# Autodesk Inventor assembly: Assembly3
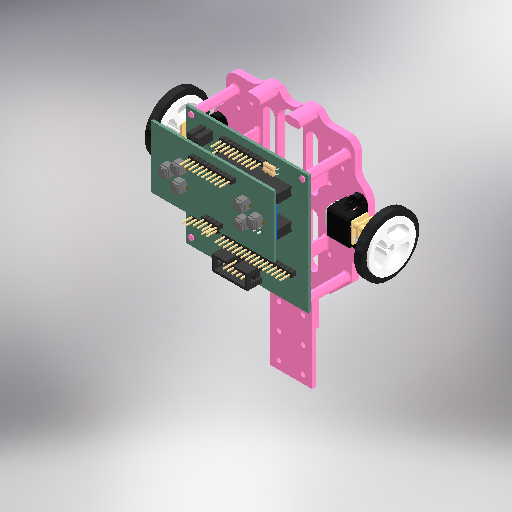
[picture p0: Inventor's stored thumbnail of the model, 512x512]
Saved by Autodesk Inventor 2025.2 (Build 292293000, 293)
## iProperties
Created: 2025-11-09
Part Number: Assembly3
Document SubType Name: Assembly
Designer: ia088
Author: ia088
## Documents named in this file (7)
- C:\Users\ia088\OneDrive\Dokumen\Prak.Robotika\board fix\Assembly3.iam
- C:\Users\ia088\OneDrive\Dokumen\Prak.Robotika\board fix\BASE_LF.ipt
- C:\Users\ia088\OneDrive\Dokumen\Prak.Robotika\board fix\motor.iam
- C:\Users\ia088\OneDrive\Dokumen\Prak.Robotika\board fix\SENSOR_3D1.iam
- C:\Users\ia088\OneDrive\Dokumen\Prak.Robotika\board fix\main_board1\main_board1\main_board1.iam
- C:\Users\ia088\OneDrive\Dokumen\Prak.Robotika\board fix\board_ctrl\board_ctrl\board_ctrl.iam
- C:\Users\ia088\OneDrive\Dokumen\Prak.Robotika\board fix\Arduino Nano\Arduino Nano\Arduino Nano.iam
## Components (7 placed, 6 different names)
1. motor:1 [sub-assembly] — Mate:4, Mate:5, Mate:6
2. motor:2 [sub-assembly] — Mate:1, Mate:2, Mate:3
3. BASE_LF:1 — Mate:1, Mate:2, Mate:3, Mate:4, Mate:5, Mate:6, Mate:7, Mate:8, Mate:9, Mate:10, Mate:11, Mate:12, Mate:13
4. SENSOR_3D1:1 [sub-assembly] — Mate:7, Mate:8, Mate:9
5. main_board1:1 [sub-assembly] — Mate:10, Mate:11, Mate:12, Mate:13, Mate:14, Flush:1, Flush:2, Flush:3, Flush:4
6. board_ctrl:1 [sub-assembly] — Mate:15, Flush:3, Flush:4
7. Arduino Nano:1 [sub-assembly] — Mate:14, Flush:1, Flush:2, Mate:15
## Relationships (19: Mate 15, Flush 4)
- Mate:1: motor:2 ↔ BASE_LF:1
- Mate:2: motor:2 ↔ BASE_LF:1
- Mate:3: motor:2 ↔ BASE_LF:1
- Mate:4: motor:1 ↔ BASE_LF:1
- Mate:5: motor:1 ↔ BASE_LF:1
- Mate:6: motor:1 ↔ BASE_LF:1
- Mate:7: BASE_LF:1 ↔ SENSOR_3D1:1
- Mate:8: BASE_LF:1 ↔ SENSOR_3D1:1
- Mate:9: BASE_LF:1 ↔ SENSOR_3D1:1
- Mate:10: BASE_LF:1 ↔ main_board1:1
- Mate:11: BASE_LF:1 ↔ main_board1:1
- Mate:12: BASE_LF:1 ↔ main_board1:1
- Mate:13: BASE_LF:1 ↔ main_board1:1
- Mate:14: main_board1:1 ↔ Arduino Nano:1
- Flush:1: main_board1:1 ↔ Arduino Nano:1
- Flush:2: main_board1:1 ↔ Arduino Nano:1
- Mate:15: board_ctrl:1 ↔ Arduino Nano:1
- Flush:3: main_board1:1 ↔ board_ctrl:1
- Flush:4: main_board1:1 ↔ board_ctrl:1
